# Autodesk Inventor assembly: HS Conveyor Axle
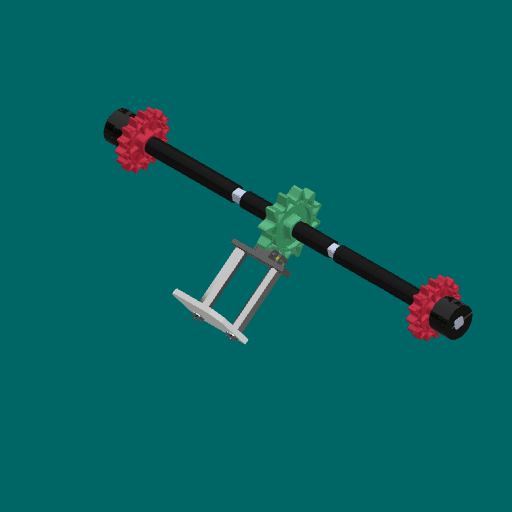
[picture p0: Inventor's stored thumbnail of the model, 512x512]
Saved by Autodesk Inventor 2025.2 (Build 292293000, 293)
## iProperties
Created: 2024-12-19
Part Number: HS Conveyor Axle
Document SubType Name: Assembly
Designer: Juan
Author: Juan
## Documents named in this file (18)
- C:\Users\colli\Documents\GitHub\ATUM-V5RC-High-Stakes-CAD\Robot\Subassemblies\HS Conveyor Axle.iam
- C:\Users\colli\Documents\GitHub\ATUM-V5RC-High-Stakes-CAD\VEX-CAD-Inventor\Motion\Shaft HS\Shaft HS\Shaft HS 10.0 in.ipt
- C:\Users\Juan\Documents\GitHub\ATUM-VRC-High-Stakes-CAD\VEX-CAD-Inventor\Motion\Shaft HS\Shaft HS.ipt
- C:\Users\colli\Documents\GitHub\ATUM-V5RC-High-Stakes-CAD\VEX-CAD-Inventor\Motion\Shaft HS\HS Spacer\HSpacer .5000.ipt
- C:\Users\Juan\Documents\GitHub\ATUM-VRC-High-Stakes-CAD\VEX-CAD-Inventor\Motion\Shaft HS\HS Spacer.ipt
- C:\Users\colli\Documents\GitHub\ATUM-V5RC-High-Stakes-CAD\VEX-CAD-Inventor\Motion\Shaft HS\HS Spacer\HSpacer .2500.ipt
- C:\Users\colli\Documents\GitHub\ATUM-V5RC-High-Stakes-CAD\VEX-CAD-Inventor\Motion\Shaft HS\HS Spacer\HSpacer .1250.ipt
- C:\Users\colli\Documents\GitHub\ATUM-V5RC-High-Stakes-CAD\VEX-CAD-Inventor\Motion\Sprockets\9P Sprocket\9P 12T Sprocket, Circle.iam
- C:\Users\Juan\Documents\GitHub\ATUM-VRC-High-Stakes-CAD\VEX-CAD-Inventor\Motion\Sprockets\9P Sprocket.iam
- C:\Users\colli\Documents\GitHub\ATUM-V5RC-High-Stakes-CAD\VEX-CAD-Inventor\Motion\Sprockets\6P Sprocket\6P 16T Sprocket, No Insert.iam
- C:\Users\Juan\Documents\GitHub\ATUM-VRC-High-Stakes-CAD\VEX-CAD-Inventor\Motion\Sprockets\6P Sprocket.iam
- C:\Users\colli\Documents\GitHub\ATUM-V5RC-High-Stakes-CAD\VEX-CAD-Inventor\Motion\Shaft HS\HS Shaft Collar.ipt
- C:\Users\colli\Documents\GitHub\ATUM-V5RC-High-Stakes-CAD\VEX-CAD-Inventor\Motion\Chain 9P\Chain Attachment Link.ipt
- C:\Users\colli\Documents\GitHub\ATUM-V5RC-High-Stakes-CAD\Hook.ipt
- C:\Users\colli\Documents\GitHub\ATUM-V5RC-High-Stakes-CAD\VEX-CAD-Inventor\Structure\Standoff\Standoff 1.50.ipt
- C:\Users\Juan\Documents\GitHub\ATUM-VRC-High-Stakes-CAD\VEX-CAD-Inventor\Structure\Standoff.ipt
- C:\Users\colli\Documents\GitHub\ATUM-V5RC-High-Stakes-CAD\VEX-CAD-Inventor\Structure\Hardware\Screw Steel - Star\SScrew Star Smooth .375.ipt
- C:\Users\Juan\Documents\GitHub\ATUM-VRC-High-Stakes-CAD\VEX-CAD-Inventor\Structure\Hardware\Screw Steel - Star.ipt
## Components (30 placed, 11 different names)
1. Shaft HS 10.0 in:1
2. HSpacer .5000:1
3. HSpacer .5000:2
4. HSpacer .5000:3 — Rigid:1
5. Chain Attachment Link:1
6. Standoff 1.50:2
7. Standoff 1.50:1
8. Hook:1 — Rigid:5, Rigid:6
9. HSpacer .5000:5
10. HSpacer .5000:6
11. HSpacer .5000:8
12. HSpacer .5000:9
13. HSpacer .5000:10 — Mate:76
14. HSpacer .5000:11 — Mate:77
15. 9P 12T Sprocket, Circle:1 [sub-assembly] — Mate:76, Mate:77
16. HSpacer .2500:14
17. HSpacer .2500:15
18. HSpacer .5000:18 — Rigid:2
19. HSpacer .1250:16
20. HSpacer .1250:17
21. 6P 16T Sprocket, No Insert:1 [sub-assembly]
22. 6P 16T Sprocket, No Insert:2 [sub-assembly]
23. HS Shaft Collar:1
24. HS Shaft Collar:2
25. HSpacer .5000:19 — Rigid:1, Rigid:4
26. HSpacer .5000:20 — Rigid:2, Rigid:3
27. HSpacer .1250:21 — Rigid:3
28. HSpacer .1250:22 — Rigid:4
29. SScrew Star Smooth .375:1 — Rigid:6
30. SScrew Star Smooth .375:2 — Rigid:5
## Relationships (70: Mate 64, WeldJoint 6)
- [Mate]: Shaft HS 10.0 in:1 ↔ HSpacer .5000:1
- [Mate]: Shaft HS 10.0 in:1 ↔ HSpacer .5000:1
- [Mate]: Shaft HS 10.0 in:1 ↔ HSpacer .5000:2
- [Mate]: Shaft HS 10.0 in:1 ↔ HSpacer .5000:2
- [Mate]: Shaft HS 10.0 in:1 ↔ HSpacer .5000:3
- [Mate]: Shaft HS 10.0 in:1 ↔ HSpacer .5000:3
- [Mate]: Shaft HS 10.0 in:1 ↔ HSpacer .5000:6
- [Mate]: Shaft HS 10.0 in:1 ↔ HSpacer .5000:6
- [Mate]: Shaft HS 10.0 in:1 ↔ HSpacer .5000:5
- [Mate]: Shaft HS 10.0 in:1 ↔ HSpacer .5000:5
- [Mate]: Shaft HS 10.0 in:1 ↔ HSpacer .5000:9
- [Mate]: Shaft HS 10.0 in:1 ↔ HSpacer .5000:9
- [Mate]: Shaft HS 10.0 in:1 ↔ HSpacer .5000:8
- [Mate]: Shaft HS 10.0 in:1 ↔ HSpacer .5000:8
- [Mate]: HSpacer .5000:3 ↔ HSpacer .5000:5
- [Mate]: HSpacer .5000:5 ↔ HSpacer .5000:8
- [Mate]: HSpacer .5000:1 ↔ HSpacer .5000:2
- [Mate]: Shaft HS 10.0 in:1 ↔ HSpacer .5000:11
- [Mate]: Shaft HS 10.0 in:1 ↔ HSpacer .5000:11
- [Mate]: HSpacer .5000:9 ↔ HSpacer .5000:11
- [Mate]: Shaft HS 10.0 in:1 ↔ HSpacer .5000:10
- [Mate]: Shaft HS 10.0 in:1 ↔ HSpacer .5000:10
- [Mate]: HSpacer .5000:6 ↔ HSpacer .5000:10
- [Mate]: Shaft HS 10.0 in:1 ↔ 9P 12T Sprocket, Circle:1
- [Mate]: Shaft HS 10.0 in:1 ↔ 9P 12T Sprocket, Circle:1
- [Mate]: Shaft HS 10.0 in:1 ↔ HSpacer .2500:14
- [Mate]: Shaft HS 10.0 in:1 ↔ HSpacer .2500:14
- [Mate]: HSpacer .5000:8 ↔ HSpacer .2500:14
- [Mate]: Shaft HS 10.0 in:1 ↔ HSpacer .2500:15
- [Mate]: Shaft HS 10.0 in:1 ↔ HSpacer .2500:15
- [Mate]: HSpacer .5000:2 ↔ HSpacer .2500:15
- [Mate]: Shaft HS 10.0 in:1 ↔ HSpacer .1250:16
- [Mate]: Shaft HS 10.0 in:1 ↔ HSpacer .1250:16
- [Mate]: HSpacer .2500:14 ↔ HSpacer .1250:16
- [Mate]: Shaft HS 10.0 in:1 ↔ HSpacer .1250:17
- [Mate]: Shaft HS 10.0 in:1 ↔ HSpacer .1250:17
- [Mate]: HSpacer .2500:15 ↔ HSpacer .1250:17
- [Mate]: Shaft HS 10.0 in:1 ↔ 6P 16T Sprocket, No Insert:1
- [Mate]: Shaft HS 10.0 in:1 ↔ 6P 16T Sprocket, No Insert:1
- [Mate]: HSpacer .1250:16 ↔ 6P 16T Sprocket, No Insert:1
- [Mate]: Shaft HS 10.0 in:1 ↔ 6P 16T Sprocket, No Insert:2
- [Mate]: Shaft HS 10.0 in:1 ↔ 6P 16T Sprocket, No Insert:2
- [Mate]: HSpacer .1250:17 ↔ 6P 16T Sprocket, No Insert:2
- [Mate]: Shaft HS 10.0 in:1 ↔ HS Shaft Collar:1
- [Mate]: Shaft HS 10.0 in:1 ↔ HS Shaft Collar:1
- [Mate]: 6P 16T Sprocket, No Insert:1 ↔ HS Shaft Collar:1
- [Mate]: Shaft HS 10.0 in:1 ↔ HS Shaft Collar:2
- [Mate]: Shaft HS 10.0 in:1 ↔ HS Shaft Collar:2
- [Mate]: 6P 16T Sprocket, No Insert:2 ↔ HS Shaft Collar:2
- [Mate]: Chain Attachment Link:1 ↔ 9P 12T Sprocket, Circle:1
- [Mate] (-2.54 mm): Chain Attachment Link:1 ↔ 9P 12T Sprocket, Circle:1
- [Mate]: Chain Attachment Link:1 ↔ Standoff 1.50:1
- [Mate]: Chain Attachment Link:1 ↔ Standoff 1.50:2
- [Mate]: Chain Attachment Link:1 ↔ Standoff 1.50:2
- [Mate] (0.1524 mm): Chain Attachment Link:1 ↔ 9P 12T Sprocket, Circle:1
- [Mate]: Chain Attachment Link:1 ↔ Standoff 1.50:1
- [Mate]: Standoff 1.50:1 ↔ Hook:1
- [Mate]: Standoff 1.50:2 ↔ Hook:1
- [Mate]: Standoff 1.50:2 ↔ Hook:1
- [Mate]: Shaft HS 10.0 in:1 ↔ HSpacer .5000:18
- [Mate]: Shaft HS 10.0 in:1 ↔ HSpacer .5000:18
- [Mate]: HSpacer .5000:1 ↔ HSpacer .5000:18
- Mate:76: HSpacer .5000:10 ↔ 9P 12T Sprocket, Circle:1
- Mate:77: HSpacer .5000:11 ↔ 9P 12T Sprocket, Circle:1
- Rigid:1 [WeldJoint]: HSpacer .5000:3 ↔ HSpacer .5000:19
- Rigid:2 [WeldJoint]: HSpacer .5000:18 ↔ HSpacer .5000:20
- Rigid:3 [WeldJoint]: HSpacer .5000:20 ↔ HSpacer .1250:21
- Rigid:4 [WeldJoint]: HSpacer .5000:19 ↔ HSpacer .1250:22
- Rigid:5 [WeldJoint]: Hook:1 ↔ SScrew Star Smooth .375:2
- Rigid:6 [WeldJoint]: Hook:1 ↔ SScrew Star Smooth .375:1
## Named parameters: d1464_d938 = 0 mm, d1465_d929 = 0 mm, d1466_d930 = -2.54 mm, d1467_d931 = 0 mm, d1468_d932 = 0 mm, d1469_d933 = 0 mm, d1470_d934 = 0.1524 mm, d1471_d935 = 0 mm, d1472_d936 = 0 mm, d1473_d937 = 0 mm
